# Autodesk Inventor assembly: Assembly
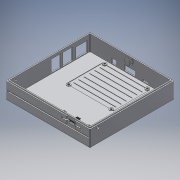
[picture p0: Inventor's stored thumbnail of the model, 180x180]
Saved by Autodesk Inventor 2018 (Build 220112000, 112)
## iProperties
Created: 2019-05-02
Part Number: Assembly
Document SubType Name: Assembly
Designer: thatg
Material: PC/ABS Plastic
Author: thatg
## Documents named in this file (5)
- C:\Users\thatg\Documents\Commodore Cube Project\Case\Assembly.iam
- C:\Users\thatg\Documents\Commodore Cube Project\Case\Tray.ipt
- C:\Users\thatg\Documents\Commodore Cube Project\Case\Dome.ipt
- C:\Users\thatg\Documents\Commodore Cube Project\Case\FloppyCover.ipt
- C:\Users\thatg\Documents\Commodore Cube Project\Case\LedCovers.ipt
## Components (4 placed, 4 different names)
1. Tray:1 — Flush:1, Flush:2, Flush:3, Flush:4
2. Dome:1 — Flush:1
3. FloppyCover:1 — Flush:2
4. LedCovers:1 — Flush:3, Flush:4
## Relationships (4: Flush 4)
- Flush:1: Tray:1 ↔ Dome:1
- Flush:2: Tray:1 ↔ FloppyCover:1
- Flush:3: Tray:1 ↔ LedCovers:1
- Flush:4: Tray:1 ↔ LedCovers:1
